# Autodesk Inventor assembly: Overall_asm
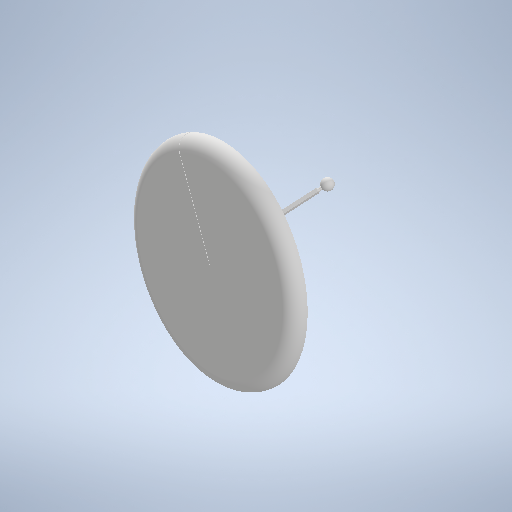
[picture p0: Inventor's stored thumbnail of the model, 512x512]
Saved by Autodesk Inventor 2025.1 (Build 291241000, 241)
## iProperties
Created: 2024-11-08
Part Number: Overall_asm
Document SubType Name: Assembly
Designer: ZOMBULLI
Author: ZOMBULLI
## Documents named in this file (5)
- C:\Users\zombulli\OneDrive - Carl Zeiss AG\Desktop\DHBW\Semester 5\mte380\Stewart Platform_new\3D-Druck\Overall_asm.iam
- C:\Users\zombulli\OneDrive - Carl Zeiss AG\Desktop\DHBW\Semester 5\mte380\Stewart Platform_new\Baseplate.ipt
- C:\Users\zombulli\OneDrive - Carl Zeiss AG\Desktop\DHBW\Semester 5\mte380\Stewart Platform_new\legs_asm_alt.iam
- C:\Users\zombulli\OneDrive - Carl Zeiss AG\Desktop\Motor\MG995 Assembly\MG995 Assembly\MG995 Assembly.iam
- C:\Users\zombulli\OneDrive - Carl Zeiss AG\Desktop\DHBW\Semester 5\mte380\Stewart Platform_new\balljoint_male.ipt
## Components (6 placed, 4 different names)
1. Baseplate:1 — Passend:1, Passend:2, Fluchtend:1, Passend:3, Passend:5
2. Baseplate:2 — Passend:3, Passend:4, Fluchtend:2, Passend:5
3. Baseplate:3 — Passend:1, Passend:2, Fluchtend:1, Passend:4, Fluchtend:2, Passend:6, Passend:7, Passend:8, Passend:10
4. legs_asm_alt:1 [sub-assembly] — Passend:9, Passend:11, Passend:12, Passend:13, Fluchtend:3, Fluchtend:4
5. MG995 Assembly:1 [sub-assembly] — Passend:6, Passend:7, Passend:8, Passend:9, Passend:10, Passend:11
6. balljoint_male:1 — Passend:12, Passend:13, Fluchtend:3, Fluchtend:4
## Relationships (17: Mate 13, Flush 4)
- Passend:1 [Mate]: Baseplate:1 ↔ Baseplate:3
- Passend:2 [Mate]: Baseplate:1 ↔ Baseplate:3
- Fluchtend:1 [Flush]: Baseplate:1 ↔ Baseplate:3
- Passend:3 [Mate]: Baseplate:1 ↔ Baseplate:2
- Passend:4 [Mate]: Baseplate:2 ↔ Baseplate:3
- Fluchtend:2 [Flush]: Baseplate:2 ↔ Baseplate:3
- Passend:5 [Mate]: Baseplate:1 ↔ Baseplate:2
- Passend:6 [Mate]: Baseplate:3 ↔ MG995 Assembly:1
- Passend:7 [Mate]: Baseplate:3 ↔ MG995 Assembly:1
- Passend:8 [Mate]: Baseplate:3 ↔ MG995 Assembly:1
- Passend:9 [Mate]: legs_asm_alt:1 ↔ MG995 Assembly:1
- Passend:10 [Mate]: Baseplate:3 ↔ MG995 Assembly:1
- Passend:11 [Mate]: legs_asm_alt:1 ↔ MG995 Assembly:1
- Passend:12 [Mate]: legs_asm_alt:1 ↔ balljoint_male:1
- Passend:13 [Mate]: legs_asm_alt:1 ↔ balljoint_male:1
- Fluchtend:3 [Flush]: legs_asm_alt:1 ↔ balljoint_male:1
- Fluchtend:4 [Flush]: legs_asm_alt:1 ↔ balljoint_male:1
